# Autodesk Inventor assembly: GPS-Compass_assembly
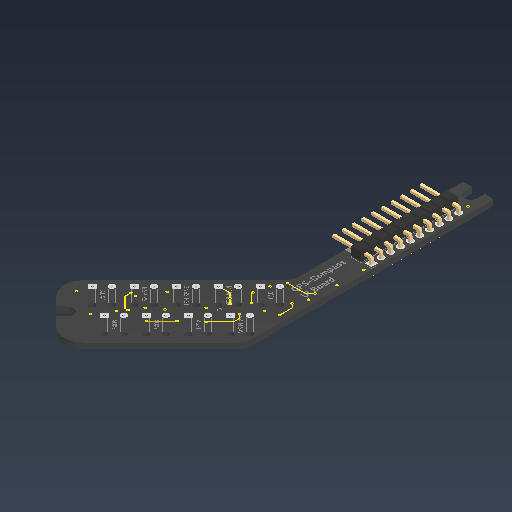
[picture p0: Inventor's stored thumbnail of the model, 512x512]
Saved by Autodesk Inventor 2026.2 (Build 302298000, 298)
## iProperties
Created: 2025-11-19
Part Number: GPS-Compass_assembly
Document SubType Name: Assembly
Designer: MenMe
Author: MenMe
## Documents named in this file (18)
- C:\Users\MenMe\GitHub\GPS-Compass\Mechanical\GPS-Compass_assembly\GPS-Compass_assembly.iam
- C:\Users\MenMe\GitHub\GPS-Compass\Mechanical\GPS-Compass_assembly\GPS-Compass_box.ipt
- C:\Users\MenMe\GitHub\GPS-Compass\Mechanical\GPS-Compass_assembly\GPS-Compass_top.ipt
- C:\Users\MenMe\GitHub\GPS-Compass\Mechanical\GPS-Compass_assembly\GPS-Compass_plexi.ipt
- C:\Users\MenMe\GitHub\GPS-Compass\Mechanical\GPS-Compass_assembly\parts\DODGE INSERT M3X4(D5-Dill4.8)\DODGE INSERT M3X4(D5-Dill4.8)\DODGE INSERT M3X4(D5-Dill4.8).ipt
- C:\Users\MenMe\GitHub\GPS-Compass\Mechanical\GPS-Compass_assembly\parts\ic184-thread\ic184-thread\ic184-thread.ipt
- C:\Users\MenMe\GitHub\GPS-Compass\Mechanical\GPS-Compass_assembly\parts\Copper Shell LED Indicator Light KL0624\Copper Shell LED Indicator Light KL0624\Copper Shell LED Indicator Light KL0624.ipt
- C:\Users\MenMe\GitHub\GPS-Compass\Mechanical\GPS-Compass_assembly\parts\EG1201\EG1201\EG1201.ipt
- C:\Users\MenMe\GitHub\GPS-Compass\Mechanical\GPS-Compass_assembly\parts\antena\antena\antena.ipt
- C:\Users\MenMe\Documents\Inventor\Content Center Files\R2026\en-US\ISO 4762(2)\ISO 4762 - M2 x 5ISO.ipt
- C:\Users\MenMe\Documents\Inventor\Content Center Files\R2026\en-US\ISO 4035(2)\ISO 4035 - M2 - ISO.ipt
- C:\Users\MenMe\GitHub\GPS-Compass\Mechanical\PCB_3D_models\GPS-Compass\GPS-Compass\GPS-Compass.ipt
- C:\Users\MenMe\GitHub\GPS-Compass\Mechanical\PCB_3D_models\GPS-Compass_UI\GPS-Compass_UI\GPS-Compass_UI.ipt
- C:\Users\MenMe\GitHub\GPS-Compass\Mechanical\PCB_3D_models\GPS-Compass_GNSS\GPS-Compass_GNSS\GPS-Compass_GNSS.ipt
- C:\Users\MenMe\GitHub\GPS-Compass\Mechanical\PCB_3D_models\GPS-Compass_Arrow\GPS-Compass_Arrow\GPS-Compass_Arrow.ipt
- C:\Users\MenMe\Documents\Inventor\Content Center Files\R2026\en-US\ISO 4762(2)\ISO 4762 - M3 x 12ISO.ipt
- C:\Users\MenMe\Documents\Inventor\Content Center Files\R2026\en-US\ISO 4762(2)\ISO 4762 - M3 x 6ISO.ipt
- C:\Users\MenMe\Documents\Inventor\Content Center Files\R2026\en-US\ISO 4762(2)\ISO 4762 - M2,5 x 6ISO.ipt
## Components (43 placed, 17 different names)
1. GPS-Compass_box:1 — Insert:7, Insert:8, Insert:9, Mate:11, Insert:10, Insert:12, Insert:15, Insert:21, Insert:23, Insert:24, Flush:5, Flush:6, Flush:7, Mate:14, Insert:27, Mate:15, Mate:16, Insert:28, Insert:29, Insert:42, Insert:43, Insert:46, Insert:47, Insert:48, Insert:49, Insert:50
2. GPS-Compass_top:1 — Mate:8, Flush:5, Flush:6, Flush:7, Mate:17, Mate:21, Mate:22, Mate:23, Mate:24, Insert:51, Insert:52, Insert:53, Insert:54, Insert:55, Insert:56
3. GPS-Compass_plexi:1 — Mate:8, Mate:17, Mate:21
4. DODGE INSERT M3X4(D5-Dill4.8):3 — Insert:7
5. DODGE INSERT M3X4(D5-Dill4.8):4 — Insert:8
6. DODGE INSERT M3X4(D5-Dill4.8):5 — Insert:9
7. DODGE INSERT M3X4(D5-Dill4.8):6 — Mate:11
8. DODGE INSERT M3X4(D5-Dill4.8):7 — Insert:10
9. DODGE INSERT M3X4(D5-Dill4.8):9 — Insert:12
10. DODGE INSERT M3X4(D5-Dill4.8):12 — Insert:15
11. DODGE INSERT M3X4(D5-Dill4.8):13
12. DODGE INSERT M3X4(D5-Dill4.8):14
13. DODGE INSERT M3X4(D5-Dill4.8):15
14. DODGE INSERT M3X4(D5-Dill4.8):16 — Insert:21
15. DODGE INSERT M3X4(D5-Dill4.8):17 — Insert:23
16. DODGE INSERT M3X4(D5-Dill4.8):18 — Insert:24
17. ic184-thread:1 — Mate:14, Insert:27
18. ic184-thread:2 — Mate:15, Insert:29
19. ic184-thread:3 — Mate:16, Insert:28
20. Copper Shell LED Indicator Light KL0624:1 — Insert:48
21. EG1201:1 — Insert:42, Insert:43, Insert:44, Insert:45
22. ISO 4762 M2 x 5:1 — Insert:44
23. ISO 4035 M2:1 — Insert:46
24. ISO 4762 M2 x 5:2 — Insert:45
25. ISO 4035 M2:2 — Insert:47
26. GPS-Compass:1 — Flush:8, Flush:9, Mate:26, Flush:10, Flush:11, Mate:27, Insert:49, Insert:50, Insert:57, Insert:58, Insert:60, Insert:62, Insert:63
27. GPS-Compass_UI:1 — Flush:8, Flush:9, Mate:26, Insert:64, Insert:65
28. GPS-Compass_GNSS:1 — Flush:10, Flush:11, Mate:27, Insert:59, Insert:61
29. GPS-Compass_Arrow:1 — Insert:51, Insert:52
30. ISO 4762 M3 x 12:1 — Insert:53
31. ISO 4762 M3 x 12:2 — Insert:54
32. ISO 4762 M3 x 12:4 — Insert:55
33. ISO 4762 M3 x 12:5 — Insert:56
34. ISO 4762 M3 x 6:1 — Insert:57
35. ISO 4762 M3 x 6:2 — Insert:58
36. ISO 4762 M3 x 6:3 — Insert:59
37. ISO 4762 M3 x 6:4 — Insert:61
38. ISO 4762 M3 x 6:5 — Insert:62
39. ISO 4762 M3 x 6:7 — Insert:63
40. ISO 4762 M3 x 6:8 — Insert:60
41. ISO 4762 M2,5 x 6:1 — Insert:64
42. ISO 4762 M2,5 x 6:2 — Insert:65
43. antena:1 — Mate:22, Mate:23, Mate:24
## Relationships (55: Insert 36, Mate 12, Flush 7)
- Mate:8: GPS-Compass_top:1 ↔ GPS-Compass_plexi:1
- Insert:7: GPS-Compass_box:1 ↔ DODGE INSERT M3X4(D5-Dill4.8):3
- Insert:8: GPS-Compass_box:1 ↔ DODGE INSERT M3X4(D5-Dill4.8):4
- Insert:9: GPS-Compass_box:1 ↔ DODGE INSERT M3X4(D5-Dill4.8):5
- Mate:11: GPS-Compass_box:1 ↔ DODGE INSERT M3X4(D5-Dill4.8):6
- Insert:10: GPS-Compass_box:1 ↔ DODGE INSERT M3X4(D5-Dill4.8):7
- Insert:12: GPS-Compass_box:1 ↔ DODGE INSERT M3X4(D5-Dill4.8):9
- Insert:15: GPS-Compass_box:1 ↔ DODGE INSERT M3X4(D5-Dill4.8):12
- Insert:21: GPS-Compass_box:1 ↔ DODGE INSERT M3X4(D5-Dill4.8):16
- Insert:23: GPS-Compass_box:1 ↔ DODGE INSERT M3X4(D5-Dill4.8):17
- Insert:24: GPS-Compass_box:1 ↔ DODGE INSERT M3X4(D5-Dill4.8):18
- Flush:5: GPS-Compass_box:1 ↔ GPS-Compass_top:1
- Flush:6: GPS-Compass_box:1 ↔ GPS-Compass_top:1
- Flush:7: GPS-Compass_box:1 ↔ GPS-Compass_top:1
- Mate:14: GPS-Compass_box:1 ↔ ic184-thread:1
- Insert:27: GPS-Compass_box:1 ↔ ic184-thread:1
- Mate:15: GPS-Compass_box:1 ↔ ic184-thread:2
- Mate:16: GPS-Compass_box:1 ↔ ic184-thread:3
- Insert:28: GPS-Compass_box:1 ↔ ic184-thread:3
- Insert:29: GPS-Compass_box:1 ↔ ic184-thread:2
- Mate:17: GPS-Compass_top:1 ↔ GPS-Compass_plexi:1
- Mate:21: GPS-Compass_top:1 ↔ GPS-Compass_plexi:1
- Insert:42: GPS-Compass_box:1 ↔ EG1201:1
- Insert:43: GPS-Compass_box:1 ↔ EG1201:1
- Mate:22: GPS-Compass_top:1 ↔ antena:1
- Mate:23: GPS-Compass_top:1 ↔ antena:1
- Mate:24: GPS-Compass_top:1 ↔ antena:1
- Insert:44: EG1201:1 ↔ ISO 4762 M2 x 5:1
- Insert:45: EG1201:1 ↔ ISO 4762 M2 x 5:2
- Insert:46: GPS-Compass_box:1 ↔ ISO 4035 M2:1
- Insert:47: GPS-Compass_box:1 ↔ ISO 4035 M2:2
- Insert:48: GPS-Compass_box:1 ↔ Copper Shell LED Indicator Light KL0624:1
- Flush:8: GPS-Compass:1 ↔ GPS-Compass_UI:1
- Flush:9: GPS-Compass:1 ↔ GPS-Compass_UI:1
- Mate:26: GPS-Compass:1 ↔ GPS-Compass_UI:1
- Flush:10: GPS-Compass:1 ↔ GPS-Compass_GNSS:1
- Flush:11: GPS-Compass:1 ↔ GPS-Compass_GNSS:1
- Mate:27: GPS-Compass:1 ↔ GPS-Compass_GNSS:1
- Insert:49: GPS-Compass_box:1 ↔ GPS-Compass:1
- Insert:50: GPS-Compass_box:1 ↔ GPS-Compass:1
- Insert:51: GPS-Compass_top:1 ↔ GPS-Compass_Arrow:1
- Insert:52: GPS-Compass_top:1 ↔ GPS-Compass_Arrow:1
- Insert:53: GPS-Compass_top:1 ↔ ISO 4762 M3 x 12:1
- Insert:54: GPS-Compass_top:1 ↔ ISO 4762 M3 x 12:2
- Insert:55: GPS-Compass_top:1 ↔ ISO 4762 M3 x 12:4
- Insert:56: GPS-Compass_top:1 ↔ ISO 4762 M3 x 12:5
- Insert:57: GPS-Compass:1 ↔ ISO 4762 M3 x 6:1
- Insert:58: GPS-Compass:1 ↔ ISO 4762 M3 x 6:2
- Insert:59: GPS-Compass_GNSS:1 ↔ ISO 4762 M3 x 6:3
- Insert:60: GPS-Compass:1 ↔ ISO 4762 M3 x 6:8
- Insert:61: GPS-Compass_GNSS:1 ↔ ISO 4762 M3 x 6:4
- Insert:62: GPS-Compass:1 ↔ ISO 4762 M3 x 6:5
- Insert:63: GPS-Compass:1 ↔ ISO 4762 M3 x 6:7
- Insert:64: GPS-Compass_UI:1 ↔ ISO 4762 M2,5 x 6:1
- Insert:65: GPS-Compass_UI:1 ↔ ISO 4762 M2,5 x 6:2
